# Autodesk Inventor assembly: aSSEMBLY2
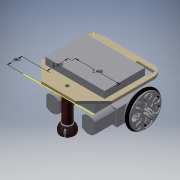
[picture p0: Inventor's stored thumbnail of the model, 180x180]
Saved by Autodesk Inventor 2016 (Build 200138000, 138)
## iProperties
Created: 2017-09-13
Part Number: aSSEMBLY2
Document SubType Name: Assembly
Designer: student
Author: student
## Documents named in this file (10)
- C:\Users\student\Documents\GitHub\Sumo-yah\aSSEMBLY2.iam
- C:\Users\student\Documents\GitHub\Sumo-yah\nEW bASE.ipt
- C:\Users\student\Documents\GitHub\Sumo-yah\Castor New.ipt
- C:\Users\student\Documents\GitHub\Sumo-yah\Motor Attach.ipt
- C:\Users\student\Documents\GitHub\Sumo-yah\Motor.ipt
- C:\Users\student\Documents\GitHub\Sumo-yah\Wheel.ipt
- C:\Users\student\Documents\GitHub\Sumo-yah\Battery.ipt
- C:\Users\student\Documents\GitHub\Sumo-yah\Ball.ipt
- C:\Users\student\Documents\GitHub\Sumo-yah\O Ring.ipt
- C:\Users\student\Documents\GitHub\Sumo-yah\Breadboard.ipt
## Components (13 placed, 9 different names)
1. nEW bASE:1 — Rigid:4, Rigid:5, Rigid:6, Rigid:7, Mate:13
2. Castor New:1 — Rigid:6, Ball:1, Mate:1, Mate:2, Mate:3, Mate:8, Mate:9, Mate:10, Mate:11, Mate:12
3. Motor Attach:1 — Rigid:1, Rigid:5
4. Motor:1 — Rigid:1, Rotational:2
5. Wheel:1 — Rotational:1, Mate:5
6. Motor Attach:2 — Rigid:3, Rigid:4
7. Motor:2 — Rigid:3, Rotational:1
8. Wheel:2 — Rotational:2, Mate:6, Mate:7
9. Battery:2 — Rigid:7
10. Ball:1 — Ball:1, Mate:1, Mate:2, Mate:3, Mate:8, Mate:9, Mate:10, Mate:11, Mate:12
11. O Ring:1 — Mate:5
12. O Ring:2 — Mate:6, Mate:7
13. Breadboard:1 — Mate:13
## Relationships (21: Mate 12, WeldJoint 6, RevoluteJoint 2, BallJoint 1)
- Rigid:1 [WeldJoint]: Motor Attach:1 ↔ Motor:1
- Rigid:3 [WeldJoint]: Motor Attach:2 ↔ Motor:2
- Rigid:4 [WeldJoint]: nEW bASE:1 ↔ Motor Attach:2
- Rigid:5 [WeldJoint]: nEW bASE:1 ↔ Motor Attach:1
- Rotational:1 [RevoluteJoint]: Wheel:1 ↔ Motor:2
- Rotational:2 [RevoluteJoint]: Motor:1 ↔ Wheel:2
- Rigid:6 [WeldJoint]: nEW bASE:1 ↔ Castor New:1
- Ball:1: Castor New:1 ↔ Ball:1
- Mate:1: Castor New:1 ↔ Ball:1
- Mate:2: Castor New:1 ↔ Ball:1
- Mate:3: Castor New:1 ↔ Ball:1
- Mate:5: Wheel:1 ↔ O Ring:1
- Mate:6: Wheel:2 ↔ O Ring:2
- Mate:7: Wheel:2 ↔ O Ring:2
- Rigid:7 [WeldJoint]: nEW bASE:1 ↔ Battery:2
- Mate:8: Castor New:1 ↔ Ball:1
- Mate:9: Castor New:1 ↔ Ball:1
- Mate:10: Castor New:1 ↔ Ball:1
- Mate:11: Castor New:1 ↔ Ball:1
- Mate:12: Castor New:1 ↔ Ball:1
- Mate:13: nEW bASE:1 ↔ Breadboard:1
